# Autodesk Inventor assembly: Longboard
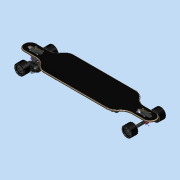
[picture p0: Inventor's stored thumbnail of the model, 180x180]
Saved by Autodesk Inventor 2015 (Build 190159000, 159)
## iProperties
Created: 2015-11-06
Part Number: Longboard
Document SubType Name: Assembly
Designer: Raphael
Author: Raphael
## Documents named in this file (6)
- \\psf\Home\Documents\electric-skateboard\CAD\Longboard.iam
- \\psf\Home\Documents\electric-skateboard\CAD\Deck.ipt
- \\psf\Home\Documents\electric-skateboard\CAD\TruckWithWheels.iam
- \\psf\Home\Documents\electric-skateboard\CAD\TruckWithMotors.iam
- \\psf\Home\Documents\electric-skateboard\CAD\ElectronicsEnclosure.iam
- \\psf\Home\Documents\electric-skateboard\CAD\BatteryPack.iam
## Components (5 placed, 5 different names)
1. Deck:1 — Mate:2, Flush:1, Mate:3, Mate:4, Mate:5, Mate:6, Tangent:1, Tangent:2, Tangent:3, Mate:7, Tangent:4, Mate:8
2. TruckWithWheels:2 [sub-assembly] — Mate:3, Mate:4, Tangent:2
3. TruckWithMotors:1 [sub-assembly] — Mate:5, Mate:6, Tangent:1
4. ElectronicsEnclosure:1 [sub-assembly] — Tangent:3, Mate:7
5. BatteryPack:1 [sub-assembly] — Tangent:4, Mate:8
## Relationships (12: Mate 7, Tangent 4, Flush 1)
- Mate:2: Deck:1
- Flush:1: Deck:1
- Mate:3: Deck:1 ↔ TruckWithWheels:2
- Mate:4: Deck:1 ↔ TruckWithWheels:2
- Mate:5: Deck:1 ↔ TruckWithMotors:1
- Mate:6: Deck:1 ↔ TruckWithMotors:1
- Tangent:1: Deck:1 ↔ TruckWithMotors:1
- Tangent:2: Deck:1 ↔ TruckWithWheels:2
- Tangent:3: Deck:1 ↔ ElectronicsEnclosure:1
- Mate:7: Deck:1 ↔ ElectronicsEnclosure:1
- Tangent:4: Deck:1 ↔ BatteryPack:1
- Mate:8: Deck:1 ↔ BatteryPack:1
